# Autodesk Inventor assembly: ceo aktuator.0001
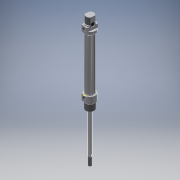
[picture p0: Inventor's stored thumbnail of the model, 180x180]
Saved by Autodesk Inventor 2019 (Build 230136000, 136)
## iProperties
Created: 2018-11-25
Part Number: ceo aktuator.0001
Document SubType Name: Assembly
Designer: aleks
Author: aleks
## Documents named in this file (5)
- C:\Users\aleks\OneDrive\Desktop\novi klip\ceo aktuator.0001.iam
- C:\Users\aleks\OneDrive\Desktop\novi klip\cilindar.ipt
- C:\Users\aleks\OneDrive\Desktop\novi klip\klipnjaca.ipt
- C:\Users\aleks\OneDrive\Desktop\novi klip\prednji deo assembly.iam
- C:\Users\aleks\OneDrive\Desktop\novi klip\zadnji deo assebly.iam
## Components (4 placed, 4 different names)
1. klipnjaca:1 — Cylindrical:1
2. cilindar:1 — Cylindrical:1, Insert:1, Insert:2
3. prednji deo assembly:1 [sub-assembly] — Insert:1, Angle:1
4. zadnji deo assebly:1 [sub-assembly] — Insert:2, Angle:1
## Relationships (4: Insert 2, CylindricalJoint 1, Angle 1)
- Cylindrical:1: klipnjaca:1 ↔ cilindar:1
- Insert:1: cilindar:1 ↔ prednji deo assembly:1
- Insert:2: cilindar:1 ↔ zadnji deo assebly:1
- Angle:1 (0 deg): prednji deo assembly:1 ↔ zadnji deo assebly:1
